# Autodesk Inventor assembly: Schieber2
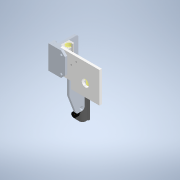
[picture p0: Inventor's stored thumbnail of the model, 180x180]
Saved by Autodesk Inventor 2022 (Build 260153000, 153)
## iProperties
Created: 2022-07-08
Part Number: Schieber2
Document SubType Name: Assembly
Designer: kaebi
Author: kaebi
## Documents named in this file (6)
- C:\Users\kaebi\OneDrive - mci4me.at\03_MCI Master\4.Semester_SS2022\Masterarbeit\Software\CAD_TeachingFactory\Schieber2.iam
- C:\Users\kaebi\OneDrive - mci4me.at\03_MCI Master\4.Semester_SS2022\Masterarbeit\Software\CAD_TeachingFactory\106.016.01_Schienenfuehrung.ipt
- C:\Users\kaebi\OneDrive - mci4me.at\03_MCI Master\4.Semester_SS2022\Masterarbeit\Software\CAD_TeachingFactory\106.034.01_Schieberelement_unten.ipt
- C:\Users\kaebi\OneDrive - mci4me.at\03_MCI Master\4.Semester_SS2022\Masterarbeit\Software\CAD_TeachingFactory\106.020.01_Winkelaufnahme_Schwert_unten.ipt
- C:\Users\kaebi\OneDrive - mci4me.at\03_MCI Master\4.Semester_SS2022\Masterarbeit\Software\CAD_TeachingFactory\106.033.01_Schwert_unten.ipt
- C:\Users\kaebi\OneDrive - mci4me.at\03_MCI Master\4.Semester_SS2022\Masterarbeit\Software\CAD_TeachingFactory\206.003.02_Kraftlimitierung.iam
## Components (6 placed, 5 different names)
1. 106.016.01_Schienenfuehrung:1
2. 106.016.01_Schienenfuehrung:2
3. 106.034.01_Schieberelement_unten:1
4. 106.020.01_Winkelaufnahme_Schwert_unten:1
5. 106.033.01_Schwert_unten:1
6. 206.003.02_Kraftlimitierung:1 [sub-assembly]
## Relationships (15: Mate 15)
- [Mate]: 106.016.01_Schienenfuehrung:2 ↔ 106.034.01_Schieberelement_unten:1
- [Mate]: 106.016.01_Schienenfuehrung:1 ↔ 106.034.01_Schieberelement_unten:1
- [Mate]: 106.034.01_Schieberelement_unten:1 ↔ 106.020.01_Winkelaufnahme_Schwert_unten:1
- [Mate]: 106.034.01_Schieberelement_unten:1 ↔ 106.020.01_Winkelaufnahme_Schwert_unten:1
- [Mate]: 106.034.01_Schieberelement_unten:1 ↔ 106.020.01_Winkelaufnahme_Schwert_unten:1
- [Mate]: 106.020.01_Winkelaufnahme_Schwert_unten:1 ↔ 106.033.01_Schwert_unten:1
- [Mate]: 106.020.01_Winkelaufnahme_Schwert_unten:1 ↔ 106.033.01_Schwert_unten:1
- [Mate]: 106.020.01_Winkelaufnahme_Schwert_unten:1 ↔ 106.033.01_Schwert_unten:1
- [Mate]: 106.034.01_Schieberelement_unten:1 ↔ 206.003.02_Kraftlimitierung:1
- [Mate]: 106.016.01_Schienenfuehrung:1 ↔ 106.034.01_Schieberelement_unten:1
- [Mate]: 106.034.01_Schieberelement_unten:1 ↔ 206.003.02_Kraftlimitierung:1
- [Mate]: 106.034.01_Schieberelement_unten:1 ↔ 206.003.02_Kraftlimitierung:1
- [Mate]: 106.016.01_Schienenfuehrung:1 ↔ 106.034.01_Schieberelement_unten:1
- [Mate]: 106.016.01_Schienenfuehrung:2 ↔ 106.034.01_Schieberelement_unten:1
- [Mate]: 106.016.01_Schienenfuehrung:2 ↔ 106.034.01_Schieberelement_unten:1
## Named parameters: d96_d84 = 0 mm, d97_d92 = 0 mm, d98_d93 = 0 mm, d99_d44 = 0 mm, d100_d45 = 0 mm, d101_d46 = 0 mm, d102_d52 = 0 mm, d103_d36 = 0 mm, d104_d37 = 0 mm, d105_d38 = 0 mm, d106_d39 = 0 mm, d107_d40 = 0 mm
